# Autodesk Inventor assembly: 1x2 Angle
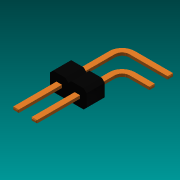
[picture p0: Inventor's stored thumbnail of the model, 180x180]
Saved by Autodesk Inventor 2015 (Build 190159000, 159)
## iProperties
Created: 2014-10-18
Part Number: 1x2 Angle
Document SubType Name: Assembly
Designer: Sawaiz Syed
Author: Sawaiz Syed
## Documents named in this file (4)
- C:\Users\Admin\SkyDrive\Classes\College\Semester 6\Research Project\Hardware\Transmitter 3D\Inventor\Radiation Dector\2.54 Breakaway\1x2 Angle.iam
- C:\Users\Admin\SkyDrive\Classes\College\Semester 6\Research Project\Hardware\Transmitter 3D\Inventor\Radiation Dector\2.54 Breakaway\Holder.ipt
- C:\Users\Admin\SkyDrive\Classes\College\Semester 6\Research Project\Hardware\Transmitter 3D\Inventor\Radiation Dector\2.54 Breakaway\PinRight1.ipt
- C:\Users\Admin\SkyDrive\Classes\College\Semester 6\Research Project\Hardware\Transmitter 3D\Inventor\Radiation Dector\2.54 Breakaway\PinRight2.ipt
## Components (4 placed, 3 different names)
1. Holder:1 — Mate:1, Mate:2, Flush:1, Mate:3, Flush:2, Flush:3
2. PinRight1:1 — Mate:1, Mate:2, Flush:1
3. Holder:2 — Mate:3, Flush:2, Flush:3, Mate:4, Mate:5, Flush:4
4. PinRight2:1 — Mate:4, Mate:5, Flush:4
## Relationships (9: Mate 5, Flush 4)
- Mate:1: Holder:1 ↔ PinRight1:1
- Mate:2: Holder:1 ↔ PinRight1:1
- Flush:1 (-6.1 mm): Holder:1 ↔ PinRight1:1
- Mate:3: Holder:1 ↔ Holder:2
- Flush:2: Holder:1 ↔ Holder:2
- Flush:3: Holder:1 ↔ Holder:2
- Mate:4: Holder:2 ↔ PinRight2:1
- Mate:5: Holder:2 ↔ PinRight2:1
- Flush:4 (-6.1 mm): Holder:2 ↔ PinRight2:1
